# Autodesk Inventor assembly: printer
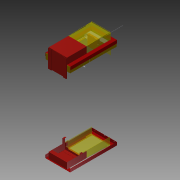
[picture p0: Inventor's stored thumbnail of the model, 180x180]
Saved by Autodesk Inventor 2014 SP2 (Build 180246200, 246)
## iProperties
Created: 2016-05-06
Part Number: printer
Document SubType Name: Assembly
Designer: cruiser
Author: cruiser
## Documents named in this file (20)
- C:\Users\cruiser\Desktop\models\3d printers\laserresin4\printer.iam
- C:\Users\cruiser\Desktop\models\3d printers\laserresin4\crane.ipt
- C:\Users\cruiser\Desktop\models\3d printers\laserresin4\carrier.ipt
- C:\Users\cruiser\Desktop\models\3d printers\laserresin4\reservoir.ipt
- C:\Users\cruiser\Desktop\models\3d printers\laserresin4\frame_inner.ipt
- C:\Users\cruiser\Desktop\models\3d printers\laserresin4\frame_lower.ipt
- C:\Users\cruiser\Desktop\models\3d printers\laserresin4\frame_face.ipt
- C:\Users\cruiser\Desktop\models\3d printers\laserresin4\door_assembly.iam
- C:\Users\cruiser\Desktop\models\3d printers\laserresin4\visor.ipt
- C:\Users\cruiser\Desktop\models\3d printers\laserresin4\frame_feet.ipt
- C:\Users\cruiser\Desktop\models\3d printers\laserresin4\bed.ipt
- C:\Users\cruiser\Desktop\models\3d printers\laserresin4\nema17.ipt
- C:\Users\cruiser\Desktop\models\3d printers\laserresin4\m8_rail.ipt
- C:\Users\cruiser\Desktop\models\3d printers\laserresin4\shf8.ipt
- C:\Users\cruiser\Desktop\models\3d printers\laserresin4\lmk8luu.ipt
- C:\Users\cruiser\Desktop\models\3d printers\laserresin4\tray.ipt
- C:\Users\cruiser\Desktop\models\3d printers\laserresin4\threaded_rod.ipt
- C:\Users\cruiser\Desktop\models\3d printers\laserresin4\subframe.ipt
- C:\Users\cruiser\Desktop\models\3d printers\laserresin4\laserholder.ipt
- C:\Users\cruiser\Desktop\models\3d printers\laserresin4\laserresin4.xlsx
## Components (25 placed, 18 different names)
1. crane:1 — Mate:1, Mate:2, Mate:16, Mate:28, Mate:29, Mate:30, Mate:33, Mate:34, Mate:46, Mate:47, Mate:48, Mate:49, Mate:50, Mate:51
2. carrier:1 — Mate:1, Mate:2, Mate:5, Mate:6, Mate:7, Mate:8, Mate:9, Mate:10, Mate:13, Mate:44, Mate:45, Mate:52, Mate:53, Mate:58, Mate:63, Mate:64
3. reservoir:1 — Mate:52, Mate:53, Mate:54, Mate:58, Mate:60, Mate:61
4. frame_inner:1 — Mate:3, Flush:1, Mate:4, Flush:2, Mate:8, Mate:9, Mate:10, Mate:14, Mate:19, Mate:21, Mate:31, Mate:32, Mate:37, Mate:38, Flush:3, Flush:4, Mate:39
5. frame_lower:1 — Mate:5, Mate:6, Mate:7, Mate:11, Mate:35, Mate:36, Mate:40, Mate:41, Mate:72, Mate:73, Mate:74
6. frame_face:1 — Mate:21, Flush:5
7. frame_face:2 — Mate:14, Mate:19, Mate:37, Flush:5, Mate:65
8. door_assembly:1 [sub-assembly] — Mate:13, Mate:18, Mate:65
9. visor:1 — Mate:3, Flush:1, Mate:32
10. visor:2 — Mate:4, Flush:2, Mate:31
11. frame_feet:1 — Mate:11, Mate:18, Mate:35, Mate:36, Mate:62
12. bed:1 — Mate:16, Mate:33, Mate:34, Mate:59
13. nema17:1 — Mate:28, Mate:29, Mate:30, Mate:56, Mate:57
14. m8_rail:1 — Mate:38, Flush:3, Mate:43
15. m8_rail:2 — Flush:4, Mate:39, Mate:42
16. shf8:1 — Mate:40, Mate:42, Mate:44
17. shf8:2 — Mate:41, Mate:43, Mate:45
18. lmk8luu:1 — Mate:46, Mate:48, Mate:50
19. lmk8luu:2 — Mate:47, Mate:49, Mate:51
20. tray:1 — Mate:54, Mate:59, Mate:60, Mate:61
21. threaded_rod:1 — Mate:56, Mate:57
22. door_assembly:2 [sub-assembly] — Mate:62, Mate:63, Mate:64
23. subframe:1 — Mate:66, Mate:67, Mate:68, Mate:69, Mate:70, Mate:71, Mate:72, Mate:73, Mate:74
24. laserholder:1 — Mate:66, Mate:68, Mate:69
25. laserholder:2 — Mate:67, Mate:70, Mate:71
## Relationships (68: Mate 63, Flush 5)
- Mate:1: crane:1 ↔ carrier:1
- Mate:2: crane:1 ↔ carrier:1
- Mate:3: frame_inner:1 ↔ visor:1
- Flush:1: frame_inner:1 ↔ visor:1
- Mate:4: frame_inner:1 ↔ visor:2
- Flush:2: frame_inner:1 ↔ visor:2
- Mate:5: carrier:1 ↔ frame_lower:1
- Mate:6: carrier:1 ↔ frame_lower:1
- Mate:7: carrier:1 ↔ frame_lower:1
- Mate:8: carrier:1 ↔ frame_inner:1
- Mate:9: carrier:1 ↔ frame_inner:1
- Mate:10: carrier:1 ↔ frame_inner:1
- Mate:11: frame_lower:1 ↔ frame_feet:1
- Mate:13: carrier:1 ↔ door_assembly:1
- Mate:14: frame_inner:1 ↔ frame_face:2
- Mate:16: crane:1 ↔ bed:1
- Mate:18: door_assembly:1 ↔ frame_feet:1
- Mate:19: frame_inner:1 ↔ frame_face:2
- Mate:21: frame_inner:1 ↔ frame_face:1
- Mate:28: crane:1 ↔ nema17:1
- Mate:29: crane:1 ↔ nema17:1
- Mate:30: crane:1 ↔ nema17:1
- Mate:31: frame_inner:1 ↔ visor:2
- Mate:32: frame_inner:1 ↔ visor:1
- Mate:33: crane:1 ↔ bed:1
- Mate:34: crane:1 ↔ bed:1
- Mate:35: frame_lower:1 ↔ frame_feet:1
- Mate:36: frame_lower:1 ↔ frame_feet:1
- Mate:37: frame_inner:1 ↔ frame_face:2
- Mate:38: frame_inner:1 ↔ m8_rail:1
- Flush:3: frame_inner:1 ↔ m8_rail:1
- Flush:4: frame_inner:1 ↔ m8_rail:2
- Mate:39: frame_inner:1 ↔ m8_rail:2
- Mate:40: frame_lower:1 ↔ shf8:1
- Mate:41: frame_lower:1 ↔ shf8:2
- Mate:42: m8_rail:2 ↔ shf8:1
- Mate:43: m8_rail:1 ↔ shf8:2
- Mate:44: carrier:1 ↔ shf8:1
- Mate:45: carrier:1 ↔ shf8:2
- Mate:46: crane:1 ↔ lmk8luu:1
- Mate:47: crane:1 ↔ lmk8luu:2
- Mate:48: crane:1 ↔ lmk8luu:1
- Mate:49: crane:1 ↔ lmk8luu:2
- Mate:50: crane:1 ↔ lmk8luu:1
- Mate:51: crane:1 ↔ lmk8luu:2
- Mate:52: carrier:1 ↔ reservoir:1
- Mate:53: carrier:1 ↔ reservoir:1
- Mate:54: reservoir:1 ↔ tray:1
- Mate:56: nema17:1 ↔ threaded_rod:1
- Mate:57: nema17:1 ↔ threaded_rod:1
- Mate:58: carrier:1 ↔ reservoir:1
- Mate:59: bed:1 ↔ tray:1
- Mate:60: reservoir:1 ↔ tray:1
- Mate:61: reservoir:1 ↔ tray:1
- Mate:62: frame_feet:1 ↔ door_assembly:2
- Mate:63: carrier:1 ↔ door_assembly:2
- Mate:64: carrier:1 ↔ door_assembly:2
- Flush:5: frame_face:1 ↔ frame_face:2
- Mate:65: frame_face:2 ↔ door_assembly:1
- Mate:66: subframe:1 ↔ laserholder:1
- Mate:67: subframe:1 ↔ laserholder:2
- Mate:68: subframe:1 ↔ laserholder:1
- Mate:69: subframe:1 ↔ laserholder:1
- Mate:70: subframe:1 ↔ laserholder:2
- Mate:71: subframe:1 ↔ laserholder:2
- Mate:72: frame_lower:1 ↔ subframe:1
- Mate:73: frame_lower:1 ↔ subframe:1
- Mate:74: frame_lower:1 ↔ subframe:1
## Named parameters: sm_thickness = 1.5875 mm, very_thick_acrylic = 9.45 mm, thick_acrylic = 5.88 mm, thin_acrylic = 3.15 mm, clear_acrylic = 3.15 mm, wood_thickness = 6.72 mm, m3_diameter = 3 mm, m4_diameter = 4 mm, m5_diameter = 5 mm, brass_insert_drill = 4 mm, m5_brass_insert_drill = 6.7 mm, m3_main_length = 14 mm, m3_main_nut_width = 5.7 mm, m3_main_nut_thickness = 2.5 mm, m3_main_extra = 1 mm, stepper_screw_space = 35 mm, stepper_shaft_diameter = 5 mm, stepper_body_diameter = 28 mm, laser_body_length = 40 mm, laser_body_diameter = 12 mm, carrier_x = 350 mm, carrier_y = 251 mm, carrier_z = 12 mm, visor_x = 257.3 mm, visor_y = 111.0625 mm, visor_overlap = 20 mm, protection_slot_length = 80 mm, protection_slot_width = 10 mm, window_z = 333.9125 mm, window_y = 92.0625 mm, window_overlap = 48 mm, acrylic_into_frame = 5 mm, door_x = 251 mm, door_z = 333.9125 mm, door_overlap = 48 mm, reservoir_x = 201 mm, reservoir_y = 201 mm, reservoir_z = 40 mm, reservoir_overlap = 20 mm, linear_bearing_spacing = 271 mm, linear_bearing_z = 400 mm, threaded_rod_z = 300 mm, motor_spacing = 337 mm, tray_border = 25 mm, tray_x = 251 mm, tray_y = 251 mm, bed_x = 150 mm, bed_y = 150 mm, bed_z = 25 mm, bed_z2 = 80 mm, stopper_diameter = 10 mm, crane_x = 330 mm, crane_y = 70 mm, crane_z = 60 mm, crane_z2 = 12 mm, end_stop_offset_x = 50 mm, end_stop_spacing = 19 mm, thumb_nut_offset_y = 0 mm, thumb_nut_diameter = 7 mm, z_min_from_center = 115 mm, frame_top_z = 385 mm, frame_bottom_z = 275 mm, frame_total_z = 661.5875 mm, frame_y = 80 mm, frame_z = 300 mm, frame_border = 46.35 mm, frame_foot_z = 12 mm, frame_tilt = 1 deg, bracket_z = 30 mm, printer_z = 289 mm, printer_from_bottom = 200 mm, middle_frame_from_bottom = 150 mm, lcd_x = 72 mm, lcd_y = 25 mm, subframe_x = 343 mm, subframe_z = 60 mm, subframe_y_offset = 27.5 mm, laser_y_offset = 19.4 mm, laser_diameter = 12 mm, laser_z_offset = 55 mm, laser_y = 15 mm, laser_z = 75 mm, laser_x = 30 mm, t_galvo_frame = 6.72 mm, galvo_frame_x = 66 mm, galvo_frame_z = 65 mm, galvo_frame_y_offset = 27.5 mm, drawer_x = 257.3 mm, drawer_y = 88.65 mm, drawer_z = 278.175 mm, drawer_z_from_bottom = 25 mm, nema17_l = 60 mm, nema17_x = 43 mm, m3_press_nut_drill = 4.5 mm, m3_head = 6 mm, m5_head = 10 mm, m5_press_nut_drill = 6.5 mm, drawer_support_from_top = 48 mm, drawer_support_overlap = 40 mm, laser_gap = 1 mm, frame_screw_from_center = 25 mm, galvo_frame_y = 20 mm, frame_magnet_offset = 20 mm, magnet_z = 50 mm, drawer_screw_z = 145 mm, drawer_screw_from_center = 54 mm, frame_face_y = 44 mm, magnet_screw_spacing = 30 mm, magnet_screw_from_edge = 10 mm, switch_spacing = 19 mm, subframe_y = 55 mm
